# Autodesk Inventor assembly: Multi-Cat-mechanical
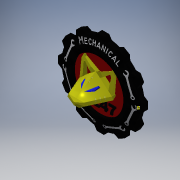
[picture p0: Inventor's stored thumbnail of the model, 180x180]
Saved by Autodesk Inventor 2016 (Build 200138000, 138)
## iProperties
Created: 2015-06-02
Part Number: Multi-Cat-mechanical
Document SubType Name: Assembly
Designer: Spooner
Author: Spooner
## Documents named in this file (10)
- C:\Users\RoksBot\Documents\Inventor\cat head\Multi-Cat-mechanical.iam
- C:\Users\RoksBot\Documents\Inventor\cat head\Background.ipt
- C:\Users\RoksBot\Documents\Inventor\cat head\Disk.ipt
- C:\Users\RoksBot\Documents\Inventor\cat head\Numbers.ipt
- C:\Users\RoksBot\Documents\Inventor\cat head\Cat.ipt
- C:\Users\RoksBot\Documents\Inventor\cat head\Eyes.ipt
- C:\Users\RoksBot\Documents\Inventor\cat head\Team Pin Mechanical.ipt
- C:\Users\RoksBot\Documents\Inventor\cat head\Team Pin Mechanical-Text.ipt
- C:\Users\RoksBot\Documents\Inventor\cat head\Team Pin Mechanical-Left Wrench.ipt
- C:\Users\RoksBot\Documents\Inventor\cat head\Team Pin Mechanical-Right Wrench.ipt
## Components (13 placed, 9 different names)
1. Background:1 — Insert:1, Angle:2, Mate:3, Mate:4, Mate:5, Mate:6
2. Disk:1 — Mate:1, Mate:2, Insert:1, Angle:1, Angle:2, Tangent:1, Angle:3, Insert:2, Angle:4
3. Numbers:1 — Mate:3, Mate:4, Mate:5
4. Cat:1 — Mate:6, Tangent:1, Angle:3, Mate:7, Mate:8, Mate:9
5. Eyes:1 — Mate:7, Mate:8, Mate:9
6. Team Pin Mechanical:1 — Insert:2, Angle:4, Mate:10, Mate:11, Mate:12, Insert:3, Mate:13, Insert:4, Mate:14, Insert:5, Mate:15, Insert:6, Mate:16, Insert:7, Mate:17, Insert:8, Mate:18
7. Team Pin Mechanical-Text:1 — Mate:10, Mate:11, Mate:12
8. Team Pin Mechanical-Left Wrench:1 — Insert:4, Mate:14
9. Team Pin Mechanical-Left Wrench:2 — Insert:5, Mate:15
10. Team Pin Mechanical-Left Wrench:3 — Insert:3, Mate:13
11. Team Pin Mechanical-Right Wrench:1 — Insert:6, Mate:16
12. Team Pin Mechanical-Right Wrench:2 — Insert:7, Mate:17
13. Team Pin Mechanical-Right Wrench:3 — Insert:8, Mate:18
## Relationships (31: Mate 18, Insert 8, Angle 4, Tangent 1)
- Mate:1: Disk:1
- Mate:2: Disk:1
- Insert:1: Background:1 ↔ Disk:1
- Angle:1 (0 deg): Disk:1
- Angle:2 (0 deg): Background:1 ↔ Disk:1
- Mate:3: Background:1 ↔ Numbers:1
- Mate:4: Background:1 ↔ Numbers:1
- Mate:5: Background:1 ↔ Numbers:1
- Mate:6: Background:1 ↔ Cat:1
- Tangent:1: Disk:1 ↔ Cat:1
- Angle:3 (0 deg): Disk:1 ↔ Cat:1
- Mate:7: Cat:1 ↔ Eyes:1
- Mate:8: Cat:1 ↔ Eyes:1
- Mate:9: Cat:1 ↔ Eyes:1
- Insert:2: Disk:1 ↔ Team Pin Mechanical:1
- Angle:4 (-90 deg): Disk:1 ↔ Team Pin Mechanical:1
- Mate:10: Team Pin Mechanical:1 ↔ Team Pin Mechanical-Text:1
- Mate:11: Team Pin Mechanical:1 ↔ Team Pin Mechanical-Text:1
- Mate:12: Team Pin Mechanical:1 ↔ Team Pin Mechanical-Text:1
- Insert:3: Team Pin Mechanical:1 ↔ Team Pin Mechanical-Left Wrench:3
- Mate:13: Team Pin Mechanical:1 ↔ Team Pin Mechanical-Left Wrench:3
- Insert:4: Team Pin Mechanical:1 ↔ Team Pin Mechanical-Left Wrench:1
- Mate:14: Team Pin Mechanical:1 ↔ Team Pin Mechanical-Left Wrench:1
- Insert:5: Team Pin Mechanical:1 ↔ Team Pin Mechanical-Left Wrench:2
- Mate:15: Team Pin Mechanical:1 ↔ Team Pin Mechanical-Left Wrench:2
- Insert:6: Team Pin Mechanical:1 ↔ Team Pin Mechanical-Right Wrench:1
- Mate:16: Team Pin Mechanical:1 ↔ Team Pin Mechanical-Right Wrench:1
- Insert:7: Team Pin Mechanical:1 ↔ Team Pin Mechanical-Right Wrench:2
- Mate:17: Team Pin Mechanical:1 ↔ Team Pin Mechanical-Right Wrench:2
- Insert:8: Team Pin Mechanical:1 ↔ Team Pin Mechanical-Right Wrench:3
- Mate:18: Team Pin Mechanical:1 ↔ Team Pin Mechanical-Right Wrench:3
